# Autodesk Inventor assembly: BG202_trajan20_21
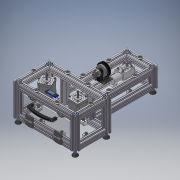
[picture p0: Inventor's stored thumbnail of the model, 180x180]
Saved by Autodesk Inventor 2022.2 (Build 262287000, 287)
## iProperties
Company: HTBLA Kaindorf
RuleStatus: InUse
Created: 2022-09-09
Part Number: BG202_trajan20_21
Project: Zeichenmaschine_v2
Material: Generisch
Description: Gerüst mit Motoren und Laufrolle
Document SubType Name: Assembly
Designer: trajan20
AfterDocNew0: iProperties-Editor_aufrufen
Author: jan
Keywords: 2021
## Documents named in this file (12)
- C:\Users\jan\Documents\DrawMachine\DrawMachineConstruction\Projekt\Zeichenmaschine_v2\BG202_trajan20_21_Zeichenmaschine_v2_Gerüst mit Motoren und Laufrolle.iam
- C:\Users\jan\Documents\DrawMachine\DrawMachineConstruction\Projekt\Zeichenmaschine_v2\BG201_trajan20_21_Zeichenmaschine_v2_gerüst_mit_platten.iam
- C:\Users\jan\Documents\DrawMachine\DrawMachineConstruction\Projekt\Zeichenmaschine_v2\step dateien\Getriebemotor.ipt
- C:\Users\jan\Documents\DrawMachine\DrawMachineConstruction\Projekt\Zeichenmaschine_v2\mot-an-s-060-005-042-l-a-aaaa.ipt
- C:\Users\jan\Documents\DrawMachine\DrawMachineConstruction\Projekt\Zeichenmaschine_v2\Normteile\de-DE\ISO 14583\ISO 14583 - M2,5x8-4.8.ipt
- C:\Users\jan\Documents\DrawMachine\DrawMachineConstruction\Projekt\Zeichenmaschine_v2\BT601_trajan20_21_Zeichenmaschine_v2_halterung.ipt
- C:\Users\jan\Documents\DrawMachine\DrawMachineConstruction\Projekt\Zeichenmaschine_v2\Normteile\de-DE\DIN 7991(2)\DIN 7991 - M3x8.ipt
- C:\Users\jan\Documents\DrawMachine\DrawMachineConstruction\Projekt\Zeichenmaschine_v2\BT602_trajan20_21_Zeichenmaschine_v2_rollte.ipt
- C:\Users\jan\Documents\DrawMachine\DrawMachineConstruction\Projekt\Zeichenmaschine_v2\Normteile\de-DE\DIN EN 24 016\DIN EN 24 016 - M12 x 55.ipt
- C:\Users\jan\Documents\DrawMachine\DrawMachineConstruction\Projekt\Zeichenmaschine_v2\Normteile\de-DE\DIN 985\DIN 985 - M12.ipt
- C:\Users\jan\Documents\DrawMachine\DrawMachineConstruction\Projekt\Zeichenmaschine_v2\Normteile\de-DE\ISO 14583\ISO 14583 - M2,5x5-4.8.ipt
- C:\Users\jan\Documents\DrawMachine\DrawMachineConstruction\Projekt\Zeichenmaschine_v2\step dateien\display_OLED_SSD1312_I2C_0.96.ipt
## Components (25 placed, 11 different names)
1. BG201_trajan20_21_Zeichenmaschine_v2_gerüst_mit_platten:1 [sub-assembly] — Passend:1, Passend:2, Winkel:1, Passend:3, Passend:4, Passend:5, Passend:6, Passend:7, Passend:8, Passend:9, Passend:10, Passend:11, Passend:12, Passend:13, Passend:14, Passend:15, Passend:16, Passend:17, Passend:18, Passend:19, Passend:20, Passend:21, Passend:22, Passend:31, Passend:32, Passend:33, Passend:35, Passend:51, Passend:52, Passend:53, Passend:54, Passend:55, Passend:56, Passend:57, Passend:58, Passend:59, Passend:60, Passend:61
2. Getriebemotor:1 — Passend:1, Passend:2, Winkel:1
3. mot-an-s-060-005-042-l-a-aaaa:1 — Passend:3, Passend:4
4. mot-an-s-060-005-042-l-a-aaaa:2 — Passend:5, Passend:6
5. BT601_trajan20_21_Zeichenmaschine_v2_halterung:1 — Passend:31, Passend:32, Passend:33, Passend:36, Passend:37, Passend:38, Passend:39, Passend:40, Passend:41, Passend:42, Passend:43, Passend:44, Passend:45, Passend:48, Passend:50
6. DIN 7991 M3x8:1 — Passend:35, Passend:36
7. DIN 7991 M3x8:2 — Passend:37, Passend:41
8. DIN 7991 M3x8:3 — Passend:38, Passend:42
9. DIN 7991 M3x8:4 — Passend:39, Passend:40
10. BT602_trajan20_21_Zeichenmaschine_v2_rollte:1 — Passend:43, Passend:44, Passend:45, Passend:47
11. DIN EN 24016 M12 x 55:1 — Passend:47, Passend:48, Passend:49
12. DIN 985 - ersetzt durch DIN EN ISO 10511 M12:1 — Passend:49, Passend:50
13. display_OLED_SSD1312_I2C_0.96:1 — Passend:59, Passend:60, Passend:61
14. Schraube ISO 14583:2011(E) M2,5x8-4.8:1 — Passend:7, Passend:8
15. Schraube ISO 14583:2011(E) M2,5x8-4.8:2 — Passend:9, Passend:10
16. Schraube ISO 14583:2011(E) M2,5x8-4.8:3 — Passend:11, Passend:21
17. Schraube ISO 14583:2011(E) M2,5x8-4.8:4 — Passend:12, Passend:22
18. Schraube ISO 14583:2011(E) M2,5x8-4.8:5 — Passend:13, Passend:19
19. Schraube ISO 14583:2011(E) M2,5x8-4.8:6 — Passend:14, Passend:20
20. Schraube ISO 14583:2011(E) M2,5x8-4.8:7 — Passend:15, Passend:17
21. Schraube ISO 14583:2011(E) M2,5x8-4.8:8 — Passend:16, Passend:18
22. Schraube ISO 14583:2011(E) M2,5x5-4.8:4 — Passend:57, Passend:58
23. Schraube ISO 14583:2011(E) M2,5x5-4.8:3 — Passend:55, Passend:56
24. Schraube ISO 14583:2011(E) M2,5x5-4.8:2 — Passend:53, Passend:54
25. Schraube ISO 14583:2011(E) M2,5x5-4.8:1 — Passend:51, Passend:52
## Relationships (52: Mate 51, Angle 1)
- Passend:1 [Mate]: BG201_trajan20_21_Zeichenmaschine_v2_gerüst_mit_platten:1 ↔ Getriebemotor:1
- Passend:2 [Mate]: BG201_trajan20_21_Zeichenmaschine_v2_gerüst_mit_platten:1 ↔ Getriebemotor:1
- Winkel:1 [Angle] (0 deg): BG201_trajan20_21_Zeichenmaschine_v2_gerüst_mit_platten:1 ↔ Getriebemotor:1
- Passend:3 [Mate]: BG201_trajan20_21_Zeichenmaschine_v2_gerüst_mit_platten:1 ↔ mot-an-s-060-005-042-l-a-aaaa:1
- Passend:4 [Mate]: BG201_trajan20_21_Zeichenmaschine_v2_gerüst_mit_platten:1 ↔ mot-an-s-060-005-042-l-a-aaaa:1
- Passend:5 [Mate]: BG201_trajan20_21_Zeichenmaschine_v2_gerüst_mit_platten:1 ↔ mot-an-s-060-005-042-l-a-aaaa:2
- Passend:6 [Mate]: BG201_trajan20_21_Zeichenmaschine_v2_gerüst_mit_platten:1 ↔ mot-an-s-060-005-042-l-a-aaaa:2
- Passend:7 [Mate]: BG201_trajan20_21_Zeichenmaschine_v2_gerüst_mit_platten:1 ↔ Schraube ISO 14583:2011(E) M2,5x8-4.8:1
- Passend:8 [Mate]: BG201_trajan20_21_Zeichenmaschine_v2_gerüst_mit_platten:1 ↔ Schraube ISO 14583:2011(E) M2,5x8-4.8:1
- Passend:9 [Mate]: BG201_trajan20_21_Zeichenmaschine_v2_gerüst_mit_platten:1 ↔ Schraube ISO 14583:2011(E) M2,5x8-4.8:2
- Passend:10 [Mate]: BG201_trajan20_21_Zeichenmaschine_v2_gerüst_mit_platten:1 ↔ Schraube ISO 14583:2011(E) M2,5x8-4.8:2
- Passend:11 [Mate]: BG201_trajan20_21_Zeichenmaschine_v2_gerüst_mit_platten:1 ↔ Schraube ISO 14583:2011(E) M2,5x8-4.8:3
- Passend:12 [Mate]: BG201_trajan20_21_Zeichenmaschine_v2_gerüst_mit_platten:1 ↔ Schraube ISO 14583:2011(E) M2,5x8-4.8:4
- Passend:13 [Mate]: BG201_trajan20_21_Zeichenmaschine_v2_gerüst_mit_platten:1 ↔ Schraube ISO 14583:2011(E) M2,5x8-4.8:5
- Passend:14 [Mate]: BG201_trajan20_21_Zeichenmaschine_v2_gerüst_mit_platten:1 ↔ Schraube ISO 14583:2011(E) M2,5x8-4.8:6
- Passend:15 [Mate]: BG201_trajan20_21_Zeichenmaschine_v2_gerüst_mit_platten:1 ↔ Schraube ISO 14583:2011(E) M2,5x8-4.8:7
- Passend:16 [Mate]: BG201_trajan20_21_Zeichenmaschine_v2_gerüst_mit_platten:1 ↔ Schraube ISO 14583:2011(E) M2,5x8-4.8:8
- Passend:17 [Mate]: BG201_trajan20_21_Zeichenmaschine_v2_gerüst_mit_platten:1 ↔ Schraube ISO 14583:2011(E) M2,5x8-4.8:7
- Passend:18 [Mate]: BG201_trajan20_21_Zeichenmaschine_v2_gerüst_mit_platten:1 ↔ Schraube ISO 14583:2011(E) M2,5x8-4.8:8
- Passend:19 [Mate]: BG201_trajan20_21_Zeichenmaschine_v2_gerüst_mit_platten:1 ↔ Schraube ISO 14583:2011(E) M2,5x8-4.8:5
- Passend:20 [Mate]: BG201_trajan20_21_Zeichenmaschine_v2_gerüst_mit_platten:1 ↔ Schraube ISO 14583:2011(E) M2,5x8-4.8:6
- Passend:21 [Mate]: BG201_trajan20_21_Zeichenmaschine_v2_gerüst_mit_platten:1 ↔ Schraube ISO 14583:2011(E) M2,5x8-4.8:3
- Passend:22 [Mate]: BG201_trajan20_21_Zeichenmaschine_v2_gerüst_mit_platten:1 ↔ Schraube ISO 14583:2011(E) M2,5x8-4.8:4
- Passend:31 [Mate]: BG201_trajan20_21_Zeichenmaschine_v2_gerüst_mit_platten:1 ↔ BT601_trajan20_21_Zeichenmaschine_v2_halterung:1
- Passend:32 [Mate]: BG201_trajan20_21_Zeichenmaschine_v2_gerüst_mit_platten:1 ↔ BT601_trajan20_21_Zeichenmaschine_v2_halterung:1
- Passend:33 [Mate]: BG201_trajan20_21_Zeichenmaschine_v2_gerüst_mit_platten:1 ↔ BT601_trajan20_21_Zeichenmaschine_v2_halterung:1
- Passend:35 [Mate]: BG201_trajan20_21_Zeichenmaschine_v2_gerüst_mit_platten:1 ↔ DIN 7991 M3x8:1
- Passend:36 [Mate]: BT601_trajan20_21_Zeichenmaschine_v2_halterung:1 ↔ DIN 7991 M3x8:1
- Passend:37 [Mate]: BT601_trajan20_21_Zeichenmaschine_v2_halterung:1 ↔ DIN 7991 M3x8:2
- Passend:38 [Mate]: BT601_trajan20_21_Zeichenmaschine_v2_halterung:1 ↔ DIN 7991 M3x8:3
- Passend:39 [Mate]: BT601_trajan20_21_Zeichenmaschine_v2_halterung:1 ↔ DIN 7991 M3x8:4
- Passend:40 [Mate]: BT601_trajan20_21_Zeichenmaschine_v2_halterung:1 ↔ DIN 7991 M3x8:4
- Passend:41 [Mate]: BT601_trajan20_21_Zeichenmaschine_v2_halterung:1 ↔ DIN 7991 M3x8:2
- Passend:42 [Mate]: BT601_trajan20_21_Zeichenmaschine_v2_halterung:1 ↔ DIN 7991 M3x8:3
- Passend:43 [Mate]: BT601_trajan20_21_Zeichenmaschine_v2_halterung:1 ↔ BT602_trajan20_21_Zeichenmaschine_v2_rollte:1
- Passend:44 [Mate] (6 mm): BT601_trajan20_21_Zeichenmaschine_v2_halterung:1 ↔ BT602_trajan20_21_Zeichenmaschine_v2_rollte:1
- Passend:45 [Mate] (24 mm): BT601_trajan20_21_Zeichenmaschine_v2_halterung:1 ↔ BT602_trajan20_21_Zeichenmaschine_v2_rollte:1
- Passend:47 [Mate]: BT602_trajan20_21_Zeichenmaschine_v2_rollte:1 ↔ DIN EN 24016 M12 x 55:1
- Passend:48 [Mate]: BT601_trajan20_21_Zeichenmaschine_v2_halterung:1 ↔ DIN EN 24016 M12 x 55:1
- Passend:49 [Mate]: DIN EN 24016 M12 x 55:1 ↔ DIN 985 - ersetzt durch DIN EN ISO 10511 M12:1
- Passend:50 [Mate]: BT601_trajan20_21_Zeichenmaschine_v2_halterung:1 ↔ DIN 985 - ersetzt durch DIN EN ISO 10511 M12:1
- Passend:51 [Mate]: BG201_trajan20_21_Zeichenmaschine_v2_gerüst_mit_platten:1 ↔ Schraube ISO 14583:2011(E) M2,5x5-4.8:1
- Passend:52 [Mate]: BG201_trajan20_21_Zeichenmaschine_v2_gerüst_mit_platten:1 ↔ Schraube ISO 14583:2011(E) M2,5x5-4.8:1
- Passend:53 [Mate]: BG201_trajan20_21_Zeichenmaschine_v2_gerüst_mit_platten:1 ↔ Schraube ISO 14583:2011(E) M2,5x5-4.8:2
- Passend:54 [Mate]: BG201_trajan20_21_Zeichenmaschine_v2_gerüst_mit_platten:1 ↔ Schraube ISO 14583:2011(E) M2,5x5-4.8:2
- Passend:55 [Mate]: BG201_trajan20_21_Zeichenmaschine_v2_gerüst_mit_platten:1 ↔ Schraube ISO 14583:2011(E) M2,5x5-4.8:3
- Passend:56 [Mate]: BG201_trajan20_21_Zeichenmaschine_v2_gerüst_mit_platten:1 ↔ Schraube ISO 14583:2011(E) M2,5x5-4.8:3
- Passend:57 [Mate]: BG201_trajan20_21_Zeichenmaschine_v2_gerüst_mit_platten:1 ↔ Schraube ISO 14583:2011(E) M2,5x5-4.8:4
- Passend:58 [Mate]: BG201_trajan20_21_Zeichenmaschine_v2_gerüst_mit_platten:1 ↔ Schraube ISO 14583:2011(E) M2,5x5-4.8:4
- Passend:59 [Mate]: BG201_trajan20_21_Zeichenmaschine_v2_gerüst_mit_platten:1 ↔ display_OLED_SSD1312_I2C_0.96:1
- Passend:60 [Mate]: BG201_trajan20_21_Zeichenmaschine_v2_gerüst_mit_platten:1 ↔ display_OLED_SSD1312_I2C_0.96:1
- Passend:61 [Mate]: BG201_trajan20_21_Zeichenmaschine_v2_gerüst_mit_platten:1 ↔ display_OLED_SSD1312_I2C_0.96:1
